# Autodesk Inventor assembly: Single door with frame3
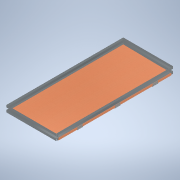
[picture p0: Inventor's stored thumbnail of the model, 180x180]
Saved by Autodesk Inventor 2021 (Build 250183000, 183)
## iProperties
Created: 2021-08-02
Part Number: Single door with frame3
Document SubType Name: Assembly
Designer: Shammy Haider
Author: Shammy Haider
## Documents named in this file (4)
- D:\Designing\Autodesk inventor\Wood Door\Single door with frame3.iam
- D:\Designing\Autodesk inventor\Wood Door\Frame3.ipt
- D:\Designing\Autodesk inventor\Wood Door\Door.ipt
- D:\Designing\Autodesk inventor\Wood Door\Hinge assembly.iam
## Components (5 placed, 3 different names)
1. Frame3:1 — Mate:1, Mate:2, Mate:3, Mate:4, Mate:5, Mate:6, Mate:7, Mate:8, Mate:9
2. Door:1 — Mate:10, Mate:11, Mate:12, Mate:13, Mate:14, Mate:15
3. Hinge assembly:1 [sub-assembly] — Mate:2, Mate:6, Mate:7, Mate:11, Mate:14
4. Hinge assembly:2 [sub-assembly] — Mate:1, Mate:8, Mate:9, Mate:12
5. Hinge assembly:3 [sub-assembly] — Mate:3, Mate:4, Mate:5, Mate:10, Mate:13, Mate:15
## Relationships (15: Mate 15)
- Mate:1: Frame3:1 ↔ Hinge assembly:2
- Mate:2: Frame3:1 ↔ Hinge assembly:1
- Mate:3: Frame3:1 ↔ Hinge assembly:3
- Mate:4: Frame3:1 ↔ Hinge assembly:3
- Mate:5: Frame3:1 ↔ Hinge assembly:3
- Mate:6: Frame3:1 ↔ Hinge assembly:1
- Mate:7: Frame3:1 ↔ Hinge assembly:1
- Mate:8: Frame3:1 ↔ Hinge assembly:2
- Mate:9: Frame3:1 ↔ Hinge assembly:2
- Mate:10: Door:1 ↔ Hinge assembly:3
- Mate:11: Door:1 ↔ Hinge assembly:1
- Mate:12: Door:1 ↔ Hinge assembly:2
- Mate:13: Door:1 ↔ Hinge assembly:3
- Mate:14: Door:1 ↔ Hinge assembly:1
- Mate:15: Door:1 ↔ Hinge assembly:3
